# Autodesk Inventor assembly: 000-A-000
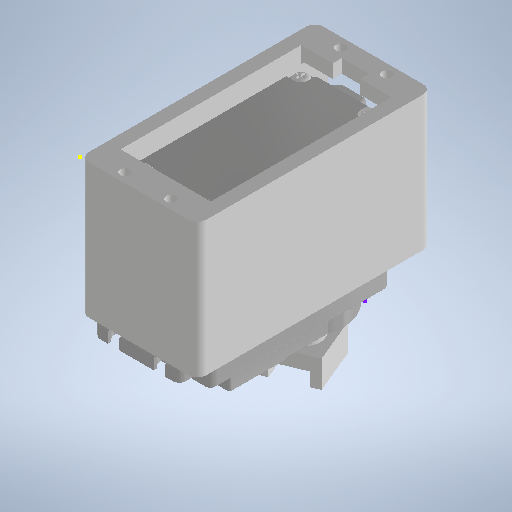
[picture p0: Inventor's stored thumbnail of the model, 512x512]
Saved by Autodesk Inventor 2025.2 (Build 292293000, 293)
## iProperties
Created: 2025-01-29
Part Number: 000-A-000
Document SubType Name: Assembly
Designer: Carriett 4
Category: <PROJECT CATAGORY>
Title: <TITLE>
Author: Carriett 4
Revision Number: A
## Documents named in this file (5)
- C:\Users\Carriett 4\OneDrive\CAD library\AILERON ASSEMBLY\ServoMechanisms\Final Servo Assembly.iam
- C:\Users\Carriett 4\OneDrive\CAD library\FLAP ASSEMBLY\HS-311-1642818408\HS-311-1642818408\HS-311-1642818408.iam
- C:\Users\Carriett 4\OneDrive\CAD library\FLAP ASSEMBLY\NewServoMount.ipt
- C:\Users\Carriett 4\OneDrive\CAD library\AILERON ASSEMBLY\ServoMechanisms\ExactServoHorn.ipt
- C:\Users\me19654\OneDrive - University of Bristol\PhD Project\005 Design (CAD and schematics)\001 Wind Tunnel\CAD Library\001-A-017 CONTRACTION ASSY.iam
## Components (3 placed, 3 different names)
1. HS-311-1642818408:1 [sub-assembly] — Rotational:1, Rotational:2
2. NewServoMount:1 — Rotational:1
3. ExactServoHorn:1 — Rotational:2
## Relationships (2: RevoluteJoint 2)
- Rotational:1 [RevoluteJoint]: HS-311-1642818408:1 ↔ NewServoMount:1
- Rotational:2 [RevoluteJoint]: HS-311-1642818408:1 ↔ ExactServoHorn:1
